# Autodesk Inventor assembly: MonterAssembly
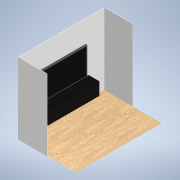
[picture p0: Inventor's stored thumbnail of the model, 180x180]
Saved by Autodesk Inventor 2020 (Build 240168000, 168)
## iProperties
Created: 2020-02-25
Part Number: MonterAssembly
Document SubType Name: Assembly
Designer: Patrik
Author: Patrik
## Documents named in this file (5)
- W:\UF-Messa-Monter\Inventor\MonterAssembly.iam
- W:\UF-Messa-Monter\Inventor\Monter.ipt
- W:\UF-Messa-Monter\Inventor\TVBänk.ipt
- W:\UF-Messa-Monter\Inventor\TV.ipt
- W:\UF-Messa-Monter\Inventor\Tavla 35x70.ipt
## Components (4 placed, 4 different names)
1. Monter:1 — Rigid:1, Rigid:2
2. TVBänk:1
3. TV:1 — Rigid:1
4. Tavla 35x70:1 — Rigid:2
## Relationships (2: WeldJoint 2)
- Rigid:1 [WeldJoint]: Monter:1 ↔ TV:1
- Rigid:2 [WeldJoint]: Monter:1 ↔ Tavla 35x70:1
